# Autodesk Inventor assembly: Jackal UGV 3D Model
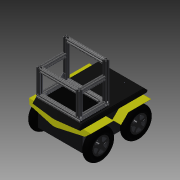
[picture p0: Inventor's stored thumbnail of the model, 180x180]
Saved by Autodesk Inventor 2015 (Build 190159000, 159)
## iProperties
Created: 2017-04-21
Part Number: Jackal UGV 3D Model
Document SubType Name: Assembly
Designer: Raghava
Author: redwards
Title: \\files\projects\ARL - US Army Research Lab\ARL02 - Jackal Dev\3-CADM\Source\Original Project\Simplified Model\Simplified Model.IGS
Description: SolidWorks IGES file using analytic representation for surfaces
Creation Date: 2015-03-12
Sending System: SolidWorks 2011
Preprocessor: SolidWorks 2011
Minimum Resolution: 0.0
Sending System Product ID: Simplified Model
Receiving System Product ID: Simplified Model
Sent Units: Millimeter
Translation Standard: IGES 5.3
Model Creation Time: 2015-03-12
Author: Raghava
## Documents named in this file (5)
- C:\Users\Raghava\Desktop\jackal_model\Jackal UGV 3D Model.iam
- C:\Users\Raghava\Desktop\jackal_model\Simplified Model Base.ipt
- C:\Users\Raghava\Desktop\jackal_model\Simplified Model Fenders.ipt
- C:\Users\Raghava\Desktop\jackal_model\Simplified Wheel.ipt
- C:\Users\Raghava\Desktop\jackal_model\8020 Components\8020_structure.iam
## Components (7 placed, 4 different names)
1. Simplified Model Base — Mate:1, Mate:2, Flush:1
2. Simplified Model Fenders
3. Simplified Wheel
4. Simplified Wheel:1
5. Simplified Wheel:2
6. Simplified Wheel:3
7. 8020_structure:1 [sub-assembly] — Mate:3, Mate:4, Flush:1
## Relationships (7: Mate 6, Flush 1)
- Mate:1: Simplified Model Base
- Mate:2: Simplified Model Base
- Mate:3: 8020_structure:1
- Mate:4: 8020_structure:1
- Mate:5
- Mate:6
- Flush:1 (5 mm): Simplified Model Base ↔ 8020_structure:1
